# Autodesk Inventor assembly: EX_ONE
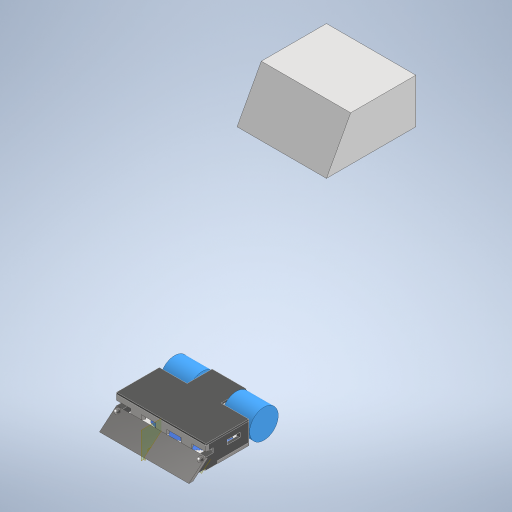
[picture p0: Inventor's stored thumbnail of the model, 512x512]
Saved by Autodesk Inventor 2023 (Build 270158000, 158)
## iProperties
Created: 2025-01-11
Part Number: EX_ONE
Document SubType Name: Assembly
Designer: kamil
Author: kamil
## Documents named in this file (14)
- C:\Users\kamil\Documents\PROJECTS - repos\EX_ONE_minisumo\mechanics\inventor_parts\EX_ONE.iam
- C:\Users\kamil\Documents\PROJECTS - repos\EX_ONE_minisumo\mechanics\inventor_parts\faulhaber_motor.ipt
- C:\Users\kamil\Documents\PROJECTS - repos\EX_ONE_minisumo\mechanics\inventor_parts\motors_mount.ipt
- C:\Users\kamil\Documents\PROJECTS - repos\EX_ONE_minisumo\mechanics\inventor_parts\kolo_tetsowe.ipt
- C:\Users\kamil\Documents\PROJECTS - repos\EX_ONE_minisumo\mechanics\inventor_parts\podstawa.ipt
- C:\Users\kamil\Documents\PROJECTS - repos\EX_ONE_minisumo\mechanics\inventor_parts\nóź.ipt
- C:\Users\kamil\Documents\PROJECTS - repos\EX_ONE_minisumo\mechanics\inventor_parts\TOF_VL53L0X (1).ipt
- C:\Users\kamil\Documents\PROJECTS - repos\EX_ONE_minisumo\mechanics\inventor_parts\pcb_pre.ipt
- C:\Users\kamil\Documents\PROJECTS - repos\EX_ONE_minisumo\mechanics\inventor_parts\minisunmo_testowe.ipt
- C:\Users\kamil\Documents\PROJECTS - repos\EX_ONE_minisumo\mechanics\inventor_parts\ściana.ipt
- C:\Users\kamil\Documents\PROJECTS - repos\EX_ONE_minisumo\mechanics\inventor_parts\ściana_MIR.ipt
- C:\Users\kamil\Documents\PROJECTS - repos\EX_ONE_minisumo\mechanics\inventor_parts\przod.ipt
- C:\Users\kamil\Documents\PROJECTS - repos\EX_ONE_minisumo\mechanics\inventor_parts\oslona.ipt
- C:\Users\kamil\Documents\PROJECTS - repos\EX_ONE_minisumo\mechanics\inventor_parts\pokrywa.ipt
## Components (20 placed, 13 different names)
1. faulhaber_motor:1 — Kątowe:1, Zestawiające:1, Zestawiające:2, Zestawiające:4, Równoległe:2
2. faulhaber_motor:2 — Kątowe:1, Zestawiające:1, Zestawiające:2, Równoległe:1, Zestawiające:3
3. motors_mount:1 — Równoległe:1, Zestawiające:3, Zestawiające:7, Równoległe:4, Zestawiające:9, Równoległe:23
4. kolo_tetsowe:1 — Zestawiające:4, Równoległe:2, Równoległe:3
5. podstawa:1 — Zestawiające:7, Równoległe:3, Równoległe:4, Równoległe:5, Równoległe:6, Równoległe:7, Równoległe:8, Zestawiające:10, Równoległe:9, Kątowe:2, Zestawiające:12, Równoległe:16, Równoległe:17, Równoległe:19, Równoległe:20, Zestawiające:15
6. nóź:1 — Równoległe:5, Równoległe:6
7. kolo_tetsowe:2 — Równoległe:7, Zestawiające:9
8. pcb_pre:1 — Równoległe:8, Zestawiające:10, Równoległe:9, Zestawiające:11, Równoległe:18
9. TOF_VL53L0X (1):1 — Zestawiające:11, Równoległe:10, Równoległe:11, Równoległe:15, Równoległe:18
10. TOF_VL53L0X (1):2 — Równoległe:11, Równoległe:15
11. TOF_VL53L0X (1):3 — Równoległe:10, Równoległe:14, Kątowe:2, Kątowe:5, Równoległe:24, Zestawiające:21, Zestawiające:23, Równoległe:26, Kątowe:8
12. TOF_VL53L0X (1):5 — Równoległe:25, Zestawiające:24, Kątowe:7, Zestawiające:26
13. TOF_VL53L0X (1):6 — Równoległe:14, Kątowe:5, Równoległe:26, Zestawiające:25, Kątowe:8, Zestawiające:27
14. minisunmo_testowe:1
15. ściana:1 — Zestawiające:12, Równoległe:16, Równoległe:17, Zestawiające:18, Równoległe:21, Zestawiające:19, Równoległe:22, Symetria:1
16. ściana_MIR:1 — Równoległe:19, Równoległe:20, Zestawiające:15, Symetria:1
17. przod:1 — Zestawiające:18, Równoległe:21, Zestawiające:19, Kątowe:6, Zestawiające:22, Zestawiające:23, Zestawiające:26, Zestawiające:27
18. oslona:1 — Równoległe:22
19. pokrywa:1 — Równoległe:23
20. TOF_VL53L0X (1):7 — Kątowe:6, Równoległe:24, Zestawiające:20, Zestawiające:22, Równoległe:25, Kątowe:7
## Relationships (51: Flush 24, Mate 20, Angle 6, Symmetry 1)
- Kątowe:1 [Angle] (180 deg): faulhaber_motor:1 ↔ faulhaber_motor:2
- Zestawiające:1 [Mate]: faulhaber_motor:1 ↔ faulhaber_motor:2
- Zestawiające:2 [Mate] (6.6 mm): faulhaber_motor:1 ↔ faulhaber_motor:2
- Równoległe:1 [Flush]: faulhaber_motor:2 ↔ motors_mount:1
- Zestawiające:3 [Mate]: faulhaber_motor:2 ↔ motors_mount:1
- Zestawiające:4 [Mate]: faulhaber_motor:1 ↔ kolo_tetsowe:1
- Równoległe:2 [Flush] (15 mm): faulhaber_motor:1 ↔ kolo_tetsowe:1
- Zestawiające:7 [Mate]: motors_mount:1 ↔ podstawa:1
- Równoległe:3 [Flush]: kolo_tetsowe:1 ↔ podstawa:1
- Równoległe:4 [Flush] (1 mm): motors_mount:1 ↔ podstawa:1
- Równoległe:5 [Flush]: podstawa:1 ↔ nóź:1
- Równoległe:6 [Flush] (3.25 mm): podstawa:1 ↔ nóź:1
- Równoległe:7 [Flush]: podstawa:1 ↔ kolo_tetsowe:2
- Zestawiające:9 [Mate]: motors_mount:1 ↔ kolo_tetsowe:2
- Równoległe:8 [Flush] (-8 mm): podstawa:1 ↔ pcb_pre:1
- Zestawiające:10 [Mate] (3 mm): podstawa:1 ↔ pcb_pre:1
- Równoległe:9 [Flush] (-2 mm): podstawa:1 ↔ pcb_pre:1
- Zestawiające:11 [Mate]: pcb_pre:1 ↔ TOF_VL53L0X (1):1
- Równoległe:10 [Flush]: TOF_VL53L0X (1):1 ↔ TOF_VL53L0X (1):3
- Równoległe:11 [Flush]: TOF_VL53L0X (1):1 ↔ TOF_VL53L0X (1):2
- Równoległe:14 [Flush]: TOF_VL53L0X (1):3 ↔ TOF_VL53L0X (1):6
- Równoległe:15 [Flush]: TOF_VL53L0X (1):1 ↔ TOF_VL53L0X (1):2
- Kątowe:2 [Angle] (15 deg): podstawa:1 ↔ TOF_VL53L0X (1):3
- Kątowe:5 [Angle] (30 deg): TOF_VL53L0X (1):3 ↔ TOF_VL53L0X (1):6
- Zestawiające:12 [Mate]: podstawa:1 ↔ ściana:1
- Równoległe:16 [Flush]: podstawa:1 ↔ ściana:1
- Równoległe:17 [Flush]: podstawa:1 ↔ ściana:1
- Równoległe:18 [Flush] (2 mm): pcb_pre:1 ↔ TOF_VL53L0X (1):1
- Równoległe:19 [Flush]: podstawa:1 ↔ ściana_MIR:1
- Równoległe:20 [Flush]: podstawa:1 ↔ ściana_MIR:1
- Zestawiające:15 [Mate]: podstawa:1 ↔ ściana_MIR:1
- Zestawiające:18 [Mate]: ściana:1 ↔ przod:1
- Równoległe:21 [Flush]: ściana:1 ↔ przod:1
- Zestawiające:19 [Mate]: ściana:1 ↔ przod:1
- Równoległe:22 [Flush]: ściana:1 ↔ oslona:1
- Równoległe:23 [Flush]: motors_mount:1 ↔ pokrywa:1
- Kątowe:6 [Angle] (-195 deg): przod:1 ↔ TOF_VL53L0X (1):7
- Równoległe:24 [Flush]: TOF_VL53L0X (1):3 ↔ TOF_VL53L0X (1):7
- Symetria:1 [Symmetry]: ściana:1 ↔ ściana_MIR:1
- Zestawiające:20 [Mate] (10 mm): TOF_VL53L0X (1):7
- Zestawiające:21 [Mate] (-10 mm): TOF_VL53L0X (1):3
- Zestawiające:22 [Mate] (2 mm): przod:1 ↔ TOF_VL53L0X (1):7
- Zestawiające:23 [Mate] (2 mm): TOF_VL53L0X (1):3 ↔ przod:1
- Równoległe:25 [Flush]: TOF_VL53L0X (1):5 ↔ TOF_VL53L0X (1):7
- Równoległe:26 [Flush]: TOF_VL53L0X (1):3 ↔ TOF_VL53L0X (1):6
- Zestawiające:24 [Mate] (34 mm): TOF_VL53L0X (1):5
- Zestawiające:25 [Mate] (-34 mm): TOF_VL53L0X (1):6
- Kątowe:7 [Angle] (30 deg): TOF_VL53L0X (1):5 ↔ TOF_VL53L0X (1):7
- Kątowe:8 [Angle] (30 deg): TOF_VL53L0X (1):3 ↔ TOF_VL53L0X (1):6
- Zestawiające:26 [Mate] (5 mm): TOF_VL53L0X (1):5 ↔ przod:1
- Zestawiające:27 [Mate] (5 mm): TOF_VL53L0X (1):6 ↔ przod:1
